# Autodesk Inventor assembly: Assembly1
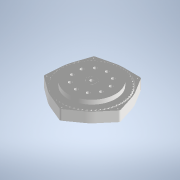
[picture p0: Inventor's stored thumbnail of the model, 180x180]
Saved by Autodesk Inventor 2022.2 (Build 262287010, 287A)
## iProperties
Created: 2022-04-27
Part Number: Assembly1
Document SubType Name: Assembly
Designer: Árni Þór Þorgeirsson
Author: Árni Þór Þorgeirsson
## Documents named in this file (8)
- C:\Users\Árni Þór Þorgeirsson\Documents\Cycloidal drive\ArniThorThorgeirsson\New folder\External Hardware\Assembly1.iam
- C:\Users\Árni Þór Þorgeirsson\Documents\Cycloidal drive\ArniThorThorgeirsson\New folder\Rotor_constructor_large_housing_output.ipt
- C:\Users\Árni Þór Þorgeirsson\Documents\Cycloidal drive\ArniThorThorgeirsson\New folder\External Hardware\skaterScrew.ipt
- C:\Users\Árni Þór Þorgeirsson\Documents\Cycloidal drive\ArniThorThorgeirsson\New folder\External Hardware\608 bearing.ipt
- C:\Users\Árni Þór Þorgeirsson\Documents\Cycloidal drive\ArniThorThorgeirsson\New folder\External Hardware\brushing.ipt
- C:\Users\Árni Þór Þorgeirsson\Documents\Cycloidal drive\ArniThorThorgeirsson\New folder\Rotor_constructor_large_rotor.ipt
- C:\Users\Árni Þór Þorgeirsson\Documents\Cycloidal drive\ArniThorThorgeirsson\New folder\External Hardware\spacer.ipt
- C:\Users\Árni Þór Þorgeirsson\Documents\Cycloidal drive\ArniThorThorgeirsson\New folder\Rotor_constructor_large_housing.ipt
## Components (38 placed, 7 different names)
1. Rotor_constructor_large_housing_output:1 — Insert:1, Insert:2, Insert:3, Insert:4, Insert:5, Mate:1, Mate:2, Mate:3, Mate:4, Mate:5, Insert:12
2. skaterScrew:1 — Insert:2, Angle:1, Tangent:1, Angle:7, Angle:8, Angle:9, Angle:10, Angle:11, Tangent:15
3. skaterScrew:2 — Insert:5, Angle:3, Tangent:4, Tangent:16, Insert:18
4. skaterScrew:3 — Insert:3, Angle:4, Tangent:3, Tangent:18
5. skaterScrew:4 — Insert:4, Angle:5, Tangent:5, Tangent:17
6. skaterScrew:5 — Insert:1, Angle:2, Tangent:2, Tangent:14
7. 608 bearing:1 — Insert:6, Angle:3, Mate:9
8. 608 bearing:2 — Insert:10, Angle:2, Mate:6
9. 608 bearing:3 — Insert:8, Angle:5, Tangent:7, Flush:1, Mate:7
10. 608 bearing:4 — Insert:7, Angle:4, Mate:8
11. 608 bearing:5 — Insert:9, Angle:1, Tangent:6, Angle:6, Mate:10
12. brushing:1 — Insert:7, Tangent:4, Mate:4, Tangent:13
13. brushing:2 — Insert:9, Tangent:3, Mate:1, Tangent:9
14. brushing:3 — Insert:8, Tangent:2, Mate:5, Tangent:12
15. brushing:4 — Insert:10, Tangent:1, Mate:2, Tangent:8
16. brushing:5 — Insert:6, Tangent:5, Mate:3, Tangent:10
17. Rotor_constructor_large_rotor:1 — Tangent:6, Angle:6, Tangent:7, Flush:1, Insert:11
18. 608 bearing:6 — Insert:11
19. 608 bearing:7 — Insert:12
20. spacer:1 — Angle:7, Tangent:8, Mate:6, Mate:15
21. spacer:2 — Angle:8, Tangent:10, Mate:9, Mate:13
22. spacer:3 — Angle:11, Tangent:12, Mate:7, Mate:12
23. spacer:4 — Angle:9, Tangent:13, Mate:8, Mate:11
24. spacer:5 — Angle:10, Tangent:9, Mate:10, Mate:14
25. 608 bearing:8 — Insert:13, Mate:13, Tangent:19, Flush:2
26. brushing:6 — Insert:13, Tangent:17
27. 608 bearing:9 — Mate:11, Tangent:20
28. brushing:7 — Tangent:16
29. 608 bearing:10 — Mate:14
30. brushing:8 — Tangent:18
31. 608 bearing:11 — Mate:15
32. brushing:9 — Tangent:15
33. 608 bearing:12 — Mate:12
34. brushing:10 — Tangent:14
35. Rotor_constructor_large_rotor:2 — Tangent:19, Tangent:20, Flush:2
36. Rotor_constructor_large_housing_output:2 — Insert:18, Cylindrical:1, Flush:3, Cylindrical:2, Flush:4
37. Rotor_constructor_large_housing:1 — Cylindrical:1, Flush:3
38. 608 bearing:13 — Cylindrical:2, Flush:4
## Relationships (69: Tangent 19, Insert 18, Mate 15, Angle 11, Flush 4, CylindricalJoint 2)
- Insert:1: Rotor_constructor_large_housing_output:1 ↔ skaterScrew:5
- Insert:2: Rotor_constructor_large_housing_output:1 ↔ skaterScrew:1
- Insert:3: Rotor_constructor_large_housing_output:1 ↔ skaterScrew:3
- Insert:4: Rotor_constructor_large_housing_output:1 ↔ skaterScrew:4
- Insert:5: Rotor_constructor_large_housing_output:1 ↔ skaterScrew:2
- Insert:6: 608 bearing:1 ↔ brushing:5
- Insert:7: 608 bearing:4 ↔ brushing:1
- Insert:8: 608 bearing:3 ↔ brushing:3
- Insert:9: 608 bearing:5 ↔ brushing:2
- Insert:10: 608 bearing:2 ↔ brushing:4
- Angle:1 (180 deg): skaterScrew:1 ↔ 608 bearing:5
- Angle:2 (180 deg): skaterScrew:5 ↔ 608 bearing:2
- Angle:3 (0 deg): skaterScrew:2 ↔ 608 bearing:1
- Angle:4 (0 deg): skaterScrew:3 ↔ 608 bearing:4
- Angle:5 (180 deg): skaterScrew:4 ↔ 608 bearing:3
- Tangent:1: skaterScrew:1 ↔ brushing:4
- Tangent:2: skaterScrew:5 ↔ brushing:3
- Tangent:3: skaterScrew:3 ↔ brushing:2
- Tangent:4: skaterScrew:2 ↔ brushing:1
- Tangent:5: skaterScrew:4 ↔ brushing:5
- Mate:1: Rotor_constructor_large_housing_output:1 ↔ brushing:2
- Mate:2: Rotor_constructor_large_housing_output:1 ↔ brushing:4
- Mate:3: Rotor_constructor_large_housing_output:1 ↔ brushing:5
- Mate:4: Rotor_constructor_large_housing_output:1 ↔ brushing:1
- Mate:5: Rotor_constructor_large_housing_output:1 ↔ brushing:3
- Tangent:6: 608 bearing:5 ↔ Rotor_constructor_large_rotor:1
- Angle:6 (0 deg): 608 bearing:5 ↔ Rotor_constructor_large_rotor:1
- Tangent:7: 608 bearing:3 ↔ Rotor_constructor_large_rotor:1
- Flush:1: 608 bearing:3 ↔ Rotor_constructor_large_rotor:1
- Insert:11: Rotor_constructor_large_rotor:1 ↔ 608 bearing:6
- Insert:12: Rotor_constructor_large_housing_output:1 ↔ 608 bearing:7
- Angle:7 (0 deg): skaterScrew:1 ↔ spacer:1
- Angle:8 (0 deg): skaterScrew:1 ↔ spacer:2
- Angle:9 (0 deg): skaterScrew:1 ↔ spacer:4
- Angle:10 (0 deg): skaterScrew:1 ↔ spacer:5
- Angle:11 (0 deg): skaterScrew:1 ↔ spacer:3
- Tangent:8: brushing:4 ↔ spacer:1
- Tangent:9: brushing:2 ↔ spacer:5
- Tangent:10: brushing:5 ↔ spacer:2
- Tangent:12: brushing:3 ↔ spacer:3
- Mate:6: 608 bearing:2 ↔ spacer:1
- Mate:7: 608 bearing:3 ↔ spacer:3
- Tangent:13: brushing:1 ↔ spacer:4
- Mate:8: 608 bearing:4 ↔ spacer:4
- Mate:9: 608 bearing:1 ↔ spacer:2
- Mate:10: 608 bearing:5 ↔ spacer:5
- Insert:13: 608 bearing:8 ↔ brushing:6
- [Insert]: 608 bearing:9 ↔ brushing:7
- [Insert]: 608 bearing:10 ↔ brushing:8
- [Insert]: 608 bearing:11 ↔ brushing:9
- [Insert]: 608 bearing:12 ↔ brushing:10
- Tangent:14: skaterScrew:5 ↔ brushing:10
- Tangent:15: skaterScrew:1 ↔ brushing:9
- Tangent:16: skaterScrew:2 ↔ brushing:7
- Tangent:17: skaterScrew:4 ↔ brushing:6
- Tangent:18: skaterScrew:3 ↔ brushing:8
- Mate:11: spacer:4 ↔ 608 bearing:9
- Mate:12: spacer:3 ↔ 608 bearing:12
- Mate:13: spacer:2 ↔ 608 bearing:8
- Mate:14: spacer:5 ↔ 608 bearing:10
- Mate:15: spacer:1 ↔ 608 bearing:11
- Tangent:19: 608 bearing:8 ↔ Rotor_constructor_large_rotor:2
- Tangent:20: 608 bearing:9 ↔ Rotor_constructor_large_rotor:2
- Flush:2: 608 bearing:8 ↔ Rotor_constructor_large_rotor:2
- Insert:18: skaterScrew:2 ↔ Rotor_constructor_large_housing_output:2
- Cylindrical:1: Rotor_constructor_large_housing_output:2 ↔ Rotor_constructor_large_housing:1
- Flush:3 (11 mm): Rotor_constructor_large_housing_output:2 ↔ Rotor_constructor_large_housing:1
- Cylindrical:2: Rotor_constructor_large_housing_output:2 ↔ 608 bearing:13
- Flush:4: Rotor_constructor_large_housing_output:2 ↔ 608 bearing:13
## Named parameters: d49_d48 = 0 mm, d50_d48 = 0 mm, d51_d48 = 0 mm, d52_d48 = 0 mm
